# Autodesk Inventor assembly: wheel_base_model
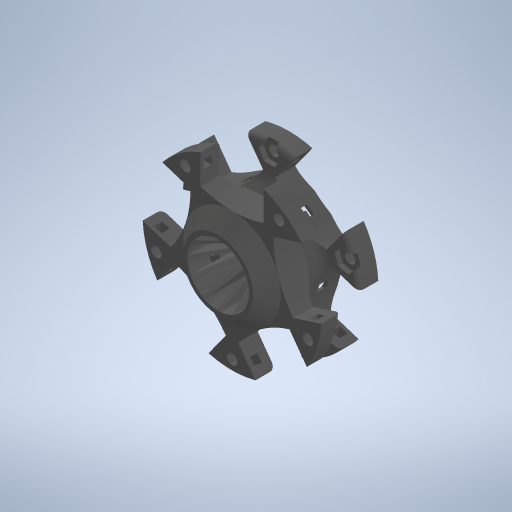
[picture p0: Inventor's stored thumbnail of the model, 512x512]
Saved by Autodesk Inventor 2024.1 (Build 281209000, 209)
## iProperties
Created: 2025-03-16
Part Number: wheel_base_model
Document SubType Name: Assembly
Designer: hibik
Author: hibik
## Documents named in this file (5)
- C:\Users\hibik\Documents\Robomech\RESCUE\ORCA\hard\simulation\wheel_base_model.iam
- C:\Users\hibik\Documents\Robomech\RESCUE\ORCA\hard\omni_wheel\wheel_body_front_outside.ipt
- C:\Users\hibik\Documents\Robomech\RESCUE\ORCA\hard\omni_wheel\wheel_body_back_inside.ipt
- C:\Users\hibik\Documents\Robomech\RESCUE\ORCA\hard\omni_wheel\wheel_body_back_outside.ipt
- C:\Users\hibik\Documents\Robomech\RESCUE\ORCA\hard\omni_wheel\wheel_body_front_inside.ipt
## Components (4 placed, 4 different names)
1. wheel_body_front_outside:1 — 挿入:1, 挿入:2, メイト:1, フラッシュ:1, メイト:2
2. wheel_body_back_inside:1 — 挿入:3, 挿入:4, 挿入:5, 挿入:6
3. wheel_body_back_outside:1 — 挿入:1, 挿入:2, 挿入:3, 挿入:4
4. wheel_body_front_inside:1 — 挿入:5, 挿入:6
## Relationships (9: Insert 6, Mate 2, Flush 1)
- 挿入:1 [Insert]: wheel_body_front_outside:1 ↔ wheel_body_back_outside:1
- 挿入:2 [Insert]: wheel_body_front_outside:1 ↔ wheel_body_back_outside:1
- 挿入:3 [Insert]: wheel_body_back_inside:1 ↔ wheel_body_back_outside:1
- 挿入:4 [Insert]: wheel_body_back_inside:1 ↔ wheel_body_back_outside:1
- 挿入:5 [Insert]: wheel_body_back_inside:1 ↔ wheel_body_front_inside:1
- 挿入:6 [Insert]: wheel_body_back_inside:1 ↔ wheel_body_front_inside:1
- メイト:1 [Mate]: wheel_body_front_outside:1
- フラッシュ:1 [Flush]: wheel_body_front_outside:1
- メイト:2 [Mate] (8.75 mm): wheel_body_front_outside:1
